# Autodesk Inventor assembly: ASY MSC 800 GILLS
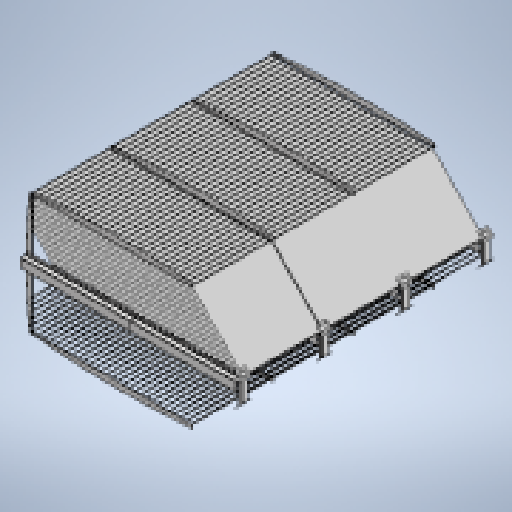
[picture p0: Inventor's stored thumbnail of the model, 512x512]
Saved by Autodesk Inventor 2025.1 (Build 291241020, 241B)
## iProperties
Created: 2024-08-31
Part Number: ASY MSC 800 GILLS
Document SubType Name: Assembly
Designer: pokla
Stock Number: ASY МОО 800 Жабры
Mass: 469810 g
Surface Area: 1.86943e+06 cm^2
Volume: 67870.7 cm^3
Density: 6.92212 g/cm^3
Author: pokla
## Documents named in this file (19)
- C:\Users\user\YandexDisk-badmisterfox\домашниий пк\Inventor\Manturovo\Manturovo_Se-clar\ASY MSC 800 gills.iam
- C:\Users\user\YandexDisk-badmisterfox\домашниий пк\Inventor\Manturovo\Manturovo_Se-clar\MSC 804 sheet gills.ipt
- C:\Users\user\YandexDisk-badmisterfox\домашниий пк\Inventor\Manturovo\Manturovo_Se-clar\MSC 810 pillar gills.ipt
- C:\Users\user\YandexDisk-badmisterfox\домашниий пк\Inventor\Manturovo\Manturovo_Se-clar\MSC 805 sheet gills.ipt
- C:\Users\user\YandexDisk-badmisterfox\домашниий пк\Inventor\Manturovo\Manturovo_Se-clar\MSC 806 sheet gills.ipt
- C:\Users\user\YandexDisk-badmisterfox\домашниий пк\Inventor\Manturovo\Manturovo_Se-clar\MSC 807 sheet gills.ipt
- C:\Users\user\YandexDisk-badmisterfox\домашниий пк\Inventor\Manturovo\Manturovo_Se-clar\MSC 808 sheet gills.ipt
- C:\Users\user\YandexDisk-badmisterfox\домашниий пк\Inventor\Manturovo\Manturovo_Se-clar\MSC 809 sheet gills.ipt
- C:\Users\user\YandexDisk-badmisterfox\домашниий пк\Inventor\Manturovo\Manturovo_Se-clar\MSC 813 wall support gills.ipt
- C:\Users\user\YandexDisk-badmisterfox\домашниий пк\Inventor\Manturovo\Manturovo_Se-clar\MSC 811 pillar gills.ipt
- C:\Users\user\YandexDisk-badmisterfox\домашниий пк\Inventor\Manturovo\Manturovo_Se-clar\MSC 814 string for sheets gills.ipt
- C:\Users\user\YandexDisk-badmisterfox\домашниий пк\Inventor\Manturovo\Manturovo_Se-clar\MSC 812 top support gills.ipt
- C:\Users\user\YandexDisk-badmisterfox\домашниий пк\Inventor\Manturovo\Manturovo_Se-clar\MSC 803 sheet gills.ipt
- C:\Users\user\YandexDisk-badmisterfox\домашниий пк\Inventor\Manturovo\Manturovo_Se-clar\ASY MSC 800.1 gills base.iam
- C:\Users\user\YandexDisk-badmisterfox\домашниий пк\Inventor\Manturovo\Manturovo_Se-clar\MSC 805 sheet gills+.ipt
- C:\Users\user\YandexDisk-badmisterfox\домашниий пк\Inventor\Manturovo\Manturovo_Se-clar\MSC 806 sheet gills+.ipt
- C:\Users\user\YandexDisk-badmisterfox\домашниий пк\Inventor\Manturovo\Manturovo_Se-clar\MSC 807 sheet gills+.ipt
- C:\Users\user\YandexDisk-badmisterfox\домашниий пк\Inventor\Manturovo\Manturovo_Se-clar\MSC 808 sheet gills+.ipt
- C:\Users\user\YandexDisk-badmisterfox\домашниий пк\Inventor\Manturovo\Manturovo_Se-clar\MSC 809 sheet gills+.ipt
## Components (297 placed, 28 different names)
1. MSC 805 sheet gills.ipt:1 — Angle:2, Tangent:8, Tangent:9, Flush:15, Flush:19, Rigid:42
2. MSC 806 sheet gills.ipt:1 — Angle:3, Tangent:10, Tangent:11, Flush:15, Flush:16, Rigid:43
3. MSC 807 sheet gills.ipt:1 — Angle:4, Tangent:12, Tangent:13, Flush:16, Flush:17, Rigid:45
4. MSC 808 sheet gills.ipt:1 — Angle:5, Tangent:17, Tangent:18, Flush:17, Flush:18, Rigid:46
5. MSC 809 sheet gills.ipt:1 — Angle:6, Tangent:19, Tangent:20, Flush:18, Rigid:47
6. MSC 814 string for sheets gills.ipt:1 — Rigid:40
7. MSC 805 sheet gills+.ipt:1 — Rigid:42
8. MSC 806 sheet gills+.ipt:1 — Rigid:43
9. MSC 807 sheet gills+.ipt:1 — Rigid:45
10. MSC 808 sheet gills+.ipt:1 — Rigid:46
11. MSC 809 sheet gills+.ipt:1 — Rigid:47
12. MSC 0203 sheet gills:2 — Rigid:53, Rigid:54
13. MSC 0204 sheet gills:2 — Rigid:54, Rigid:55
14. MSC 0205 sheet gills:2 — Rigid:55, Rigid:56
15. MSC 0206 sheet gills:2 — Rigid:56, Rigid:57
16. MSC 0207 sheet gills:2 — Rigid:57
17. MSC 0103 sheet gills:2
18. MSC 0104 sheet gills:2
19. MSC 0105 sheet gills:2
20. MSC 0106 sheet gills:2
21. MSC 0107 sheet gills:2
22. MSC 814 string for sheets gills.ipt:2 — Rigid:24
23. MSC 814 string for sheets gills.ipt:3
24. MSC 814 string for sheets gills.ipt:4
25. MSC 814 string for sheets gills.ipt:5
26. MSC 814 string for sheets gills.ipt:6
27. MSC 814 string for sheets gills.ipt:7
28. MSC 814 string for sheets gills.ipt:8 — Rigid:12
29. MSC 803 sheet gills.ipt:1 — Rigid:33, Angle:2, Angle:3, Angle:4, Angle:5, Angle:6, Tangent:14, Tangent:15, Tangent:16, Flush:19, Flush:24
30. MSC 804 sheet gills.ipt:1 — Rigid:33
31. MSC 814 string for sheets gills.ipt:9 — Rotational:1
32. MSC 814 string for sheets gills.ipt:10 — Rotational:2, Tangent:23
33. MSC 814 string for sheets gills.ipt:11 — Rotational:3, Tangent:21, Tangent:22
34. MSC 803 sheet gills.ipt:2 — Tangent:21, Tangent:23, Flush:24
35. MSC 804 sheet gills.ipt:2 — Tangent:22
36. MSC 814 string for sheets gills.ipt:12
37. MSC 803 sheet gills.ipt:3
38. MSC 804 sheet gills.ipt:3
39. MSC 814 string for sheets gills.ipt:13
40. MSC 814 string for sheets gills.ipt:14
41. MSC 814 string for sheets gills.ipt:15
42. MSC 803 sheet gills.ipt:4
43. MSC 804 sheet gills.ipt:4
44. MSC 814 string for sheets gills.ipt:16
45. MSC 803 sheet gills.ipt:5
46. MSC 804 sheet gills.ipt:5
47. MSC 814 string for sheets gills.ipt:17
48. MSC 814 string for sheets gills.ipt:18
49. MSC 814 string for sheets gills.ipt:19
50. MSC 803 sheet gills.ipt:6
51. MSC 804 sheet gills.ipt:6
52. MSC 814 string for sheets gills.ipt:20
53. MSC 803 sheet gills.ipt:7
54. MSC 804 sheet gills.ipt:7
55. MSC 814 string for sheets gills.ipt:21
56. MSC 814 string for sheets gills.ipt:22
57. MSC 814 string for sheets gills.ipt:23
58. MSC 803 sheet gills.ipt:8
59. MSC 804 sheet gills.ipt:8
60. MSC 814 string for sheets gills.ipt:24
61. MSC 803 sheet gills.ipt:9
62. MSC 804 sheet gills.ipt:9
63. MSC 814 string for sheets gills.ipt:25
64. MSC 814 string for sheets gills.ipt:26
65. MSC 814 string for sheets gills.ipt:27
66. MSC 803 sheet gills.ipt:10
67. MSC 804 sheet gills.ipt:10
68. MSC 814 string for sheets gills.ipt:28
69. MSC 803 sheet gills.ipt:11
70. MSC 804 sheet gills.ipt:11
71. MSC 814 string for sheets gills.ipt:29
72. MSC 814 string for sheets gills.ipt:30
73. MSC 814 string for sheets gills.ipt:31
74. MSC 803 sheet gills.ipt:12
75. MSC 804 sheet gills.ipt:12
76. MSC 814 string for sheets gills.ipt:32
77. MSC 803 sheet gills.ipt:13
78. MSC 804 sheet gills.ipt:13
79. MSC 814 string for sheets gills.ipt:33
80. MSC 814 string for sheets gills.ipt:34
81. MSC 814 string for sheets gills.ipt:35
82. MSC 803 sheet gills.ipt:14
83. MSC 804 sheet gills.ipt:14
84. MSC 814 string for sheets gills.ipt:36
85. MSC 803 sheet gills.ipt:15
86. MSC 804 sheet gills.ipt:15
87. MSC 814 string for sheets gills.ipt:37
88. MSC 814 string for sheets gills.ipt:38
89. MSC 814 string for sheets gills.ipt:39
90. MSC 803 sheet gills.ipt:16
91. MSC 804 sheet gills.ipt:16
92. MSC 814 string for sheets gills.ipt:40
93. MSC 803 sheet gills.ipt:17
94. MSC 804 sheet gills.ipt:17
95. MSC 814 string for sheets gills.ipt:41
96. MSC 814 string for sheets gills.ipt:42
97. MSC 814 string for sheets gills.ipt:43
98. MSC 803 sheet gills.ipt:18
99. MSC 804 sheet gills.ipt:18
100. MSC 814 string for sheets gills.ipt:44
101. MSC 803 sheet gills.ipt:19
102. MSC 804 sheet gills.ipt:19
103. MSC 814 string for sheets gills.ipt:45
104. MSC 814 string for sheets gills.ipt:46
105. MSC 814 string for sheets gills.ipt:47
106. MSC 803 sheet gills.ipt:20
107. MSC 804 sheet gills.ipt:20
108. MSC 814 string for sheets gills.ipt:48
109. MSC 803 sheet gills.ipt:21
110. MSC 804 sheet gills.ipt:21
111. MSC 814 string for sheets gills.ipt:49
112. MSC 814 string for sheets gills.ipt:50
113. MSC 814 string for sheets gills.ipt:51
114. MSC 803 sheet gills.ipt:22
115. MSC 804 sheet gills.ipt:22
116. MSC 814 string for sheets gills.ipt:52
117. MSC 803 sheet gills.ipt:23
118. MSC 804 sheet gills.ipt:23
119. MSC 814 string for sheets gills.ipt:53
120. MSC 814 string for sheets gills.ipt:54
121. MSC 814 string for sheets gills.ipt:55
122. MSC 803 sheet gills.ipt:24
123. MSC 804 sheet gills.ipt:24
124. MSC 814 string for sheets gills.ipt:56
125. MSC 803 sheet gills.ipt:25
126. MSC 804 sheet gills.ipt:25
127. MSC 814 string for sheets gills.ipt:57
128. MSC 814 string for sheets gills.ipt:58
129. MSC 814 string for sheets gills.ipt:59
130. MSC 803 sheet gills.ipt:26
131. MSC 804 sheet gills.ipt:26
132. MSC 814 string for sheets gills.ipt:60
133. MSC 803 sheet gills.ipt:27
134. MSC 804 sheet gills.ipt:27
135. MSC 814 string for sheets gills.ipt:61
136. MSC 814 string for sheets gills.ipt:62
137. MSC 814 string for sheets gills.ipt:63
138. MSC 803 sheet gills.ipt:28
139. MSC 804 sheet gills.ipt:28
140. MSC 814 string for sheets gills.ipt:64
141. MSC 803 sheet gills.ipt:29
142. MSC 804 sheet gills.ipt:29
143. MSC 814 string for sheets gills.ipt:65
144. MSC 814 string for sheets gills.ipt:66
145. MSC 814 string for sheets gills.ipt:67
146. MSC 803 sheet gills.ipt:30
147. MSC 804 sheet gills.ipt:30
148. MSC 814 string for sheets gills.ipt:68
149. MSC 803 sheet gills.ipt:31
150. MSC 804 sheet gills.ipt:31
151. MSC 814 string for sheets gills.ipt:69
152. MSC 814 string for sheets gills.ipt:70
153. MSC 814 string for sheets gills.ipt:71
154. MSC 803 sheet gills.ipt:32
155. MSC 804 sheet gills.ipt:32
156. MSC 814 string for sheets gills.ipt:72
157. MSC 803 sheet gills.ipt:33
158. MSC 804 sheet gills.ipt:33
159. MSC 814 string for sheets gills.ipt:73
160. MSC 814 string for sheets gills.ipt:74
161. MSC 814 string for sheets gills.ipt:75
162. MSC 803 sheet gills.ipt:34
163. MSC 804 sheet gills.ipt:34
164. MSC 814 string for sheets gills.ipt:76
165. MSC 803 sheet gills.ipt:35
166. MSC 804 sheet gills.ipt:35
167. MSC 814 string for sheets gills.ipt:77
168. MSC 814 string for sheets gills.ipt:78
169. MSC 814 string for sheets gills.ipt:79
170. MSC 803 sheet gills.ipt:36
171. MSC 804 sheet gills.ipt:36
172. MSC 814 string for sheets gills.ipt:80
173. MSC 803 sheet gills.ipt:37
174. MSC 804 sheet gills.ipt:37
175. MSC 814 string for sheets gills.ipt:81
176. MSC 814 string for sheets gills.ipt:82
177. MSC 814 string for sheets gills.ipt:83
178. MSC 803 sheet gills.ipt:38
179. MSC 804 sheet gills.ipt:38
180. MSC 814 string for sheets gills.ipt:84
181. MSC 803 sheet gills.ipt:39
182. MSC 804 sheet gills.ipt:39
183. MSC 814 string for sheets gills.ipt:85
184. MSC 814 string for sheets gills.ipt:86
185. MSC 814 string for sheets gills.ipt:87
186. MSC 803 sheet gills.ipt:40
187. MSC 804 sheet gills.ipt:40
188. MSC 814 string for sheets gills.ipt:88
189. MSC 803 sheet gills.ipt:41
190. MSC 804 sheet gills.ipt:41
191. MSC 814 string for sheets gills.ipt:89
192. MSC 814 string for sheets gills.ipt:90
193. MSC 814 string for sheets gills.ipt:91
194. MSC 803 sheet gills.ipt:42
195. MSC 804 sheet gills.ipt:42
196. MSC 814 string for sheets gills.ipt:92
197. MSC 803 sheet gills.ipt:43
198. MSC 804 sheet gills.ipt:43
199. MSC 814 string for sheets gills.ipt:93
200. MSC 814 string for sheets gills.ipt:94
201. MSC 814 string for sheets gills.ipt:95
202. MSC 803 sheet gills.ipt:44
203. MSC 804 sheet gills.ipt:44
204. MSC 814 string for sheets gills.ipt:96
205. MSC 803 sheet gills.ipt:45
206. MSC 804 sheet gills.ipt:45
207. MSC 814 string for sheets gills.ipt:97
208. MSC 814 string for sheets gills.ipt:98
209. MSC 814 string for sheets gills.ipt:99
210. MSC 803 sheet gills.ipt:46
211. MSC 804 sheet gills.ipt:46
212. MSC 814 string for sheets gills.ipt:100
213. MSC 803 sheet gills.ipt:47
214. MSC 804 sheet gills.ipt:47
215. MSC 814 string for sheets gills.ipt:101
216. MSC 814 string for sheets gills.ipt:102
217. MSC 814 string for sheets gills.ipt:103
218. MSC 803 sheet gills.ipt:48
219. MSC 804 sheet gills.ipt:48
220. MSC 814 string for sheets gills.ipt:104
221. MSC 803 sheet gills.ipt:49
222. MSC 804 sheet gills.ipt:49
223. MSC 814 string for sheets gills.ipt:105
224. MSC 814 string for sheets gills.ipt:106
225. MSC 814 string for sheets gills.ipt:107
226. MSC 803 sheet gills.ipt:50
227. MSC 804 sheet gills.ipt:50
228. MSC 814 string for sheets gills.ipt:108
229. MSC 803 sheet gills.ipt:51
230. MSC 804 sheet gills.ipt:51
231. MSC 814 string for sheets gills.ipt:109
232. MSC 814 string for sheets gills.ipt:110
233. MSC 814 string for sheets gills.ipt:111
234. MSC 803 sheet gills.ipt:52
235. MSC 804 sheet gills.ipt:52
236. MSC 814 string for sheets gills.ipt:112
237. MSC 803 sheet gills.ipt:53
238. MSC 804 sheet gills.ipt:53
239. MSC 814 string for sheets gills.ipt:113
240. MSC 814 string for sheets gills.ipt:114
241. MSC 814 string for sheets gills.ipt:115
242. MSC 803 sheet gills.ipt:54
243. MSC 804 sheet gills.ipt:54
244. MSC 814 string for sheets gills.ipt:116
245. MSC 803 sheet gills.ipt:55
246. MSC 804 sheet gills.ipt:55
247. MSC 814 string for sheets gills.ipt:117
248. MSC 814 string for sheets gills.ipt:118
249. MSC 814 string for sheets gills.ipt:119
250. MSC 803 sheet gills.ipt:56
251. MSC 804 sheet gills.ipt:56
252. MSC 814 string for sheets gills.ipt:120
253. MSC 803 sheet gills.ipt:57
254. MSC 804 sheet gills.ipt:57
255. MSC 814 string for sheets gills.ipt:121
256. MSC 814 string for sheets gills.ipt:122
257. MSC 814 string for sheets gills.ipt:123
258. MSC 803 sheet gills.ipt:58 — Rigid:53
259. MSC 804 sheet gills.ipt:58
260. MSC 813 wall support gills.ipt:1 — Rigid:12, Rigid:30, Tangent:14, Tangent:15
261. MSC 812 top support gills.ipt:1 — Rigid:28, Rigid:30, Tangent:8, Tangent:9, Tangent:10, Tangent:11, Tangent:12, Tangent:13, Tangent:17, Tangent:18, Tangent:19, Tangent:20, Rigid:40, Rigid:44
262. MSC 811 pillar gills.ipt:1 — Rigid:28, Rigid:29
263. MSC 812 top support gills.ipt:2 — Rigid:24, Rigid:29, Rigid:31
264. MSC 813 wall support gills.ipt:2 — Rigid:31, Rotational:3
265. MSC 810 pillar gills.ipt:1 — Rotational:1, Rotational:2, Tangent:16
266. ASY MSC 800.1 gills base.iam:1 [sub-assembly]
267. MSC 813 wall support gills.ipt:3
268. MSC 812 top support gills.ipt:3
269. MSC 811 pillar gills.ipt:2
270. MSC 812 top support gills.ipt:4
271. MSC 813 wall support gills.ipt:4
272. MSC 810 pillar gills.ipt:2
273. ASY MSC 800.1 gills base.iam:2 [sub-assembly]
274. MSC 813 wall support gills.ipt:5
275. MSC 812 top support gills.ipt:5
276. MSC 811 pillar gills.ipt:3
277. MSC 812 top support gills.ipt:6
278. MSC 813 wall support gills.ipt:6
279. MSC 810 pillar gills.ipt:3
280. ASY MSC 800.1 gills base.iam:3 [sub-assembly]
281. MSC 813 wall support gills.ipt:7
282. MSC 812 top support gills.ipt:7
283. MSC 811 pillar gills.ipt:4 — Rotational:4
284. MSC 812 top support gills.ipt:8
285. MSC 813 wall support gills.ipt:8
286. MSC 810 pillar gills.ipt:4
287. ASY MSC 800.1 gills base.iam:4 [sub-assembly]
288. MSC 814 string for sheets gills.ipt:124 — Rotational:4
289. MSC 814 string for sheets gills.ipt:125
290. MSC 814 string for sheets gills.ipt:126
291. MSC 814 string for sheets gills.ipt:127
292. MSC 814 string for sheets gills.ipt:128
293. MSC 814 string for sheets gills.ipt:129 — Rigid:44
294. MSC 814 string for sheets gills.ipt:130
295. MSC 814 string for sheets gills.ipt:131
296. MSC 814 string for sheets gills.ipt:132
297. MSC 814 string for sheets gills.ipt:133
## Component patterns: (6 elements, first: MSC 814 string for sheets gills.ipt:2), (29 elements, first: MSC 814 string for sheets gills.ipt:8 + MSC 803 sheet gills.ipt:1 + MSC 804 sheet gills.ipt:1 + MSC 814 string for sheets gills.ipt:9 + MSC 814 string for sheets gills.ipt:10 + MSC 814 string for sheets gills.ipt:11 + MSC 803 sheet gills.ipt:2 + MSC 804 sheet gills.ipt:2), (4 elements, first: MSC 813 wall support gills.ipt:1 + MSC 812 top support gills.ipt:1 + MSC 811 pillar gills.ipt:1 + MSC 812 top support gills.ipt:2 + MSC 813 wall support gills.ipt:2 + MSC 810 pillar gills.ipt:1 + ASY MSC 800.1 gills base.iam:1), (5 elements, first: MSC 814 string for sheets gills.ipt:124), (5 elements, first: MSC 814 string for sheets gills.ipt:129)
## Relationships (64: WeldJoint 26, Tangent 16, Flush 10, Angle 5, RevoluteJoint 4, Mate 3)
- [WeldJoint]: MSC 811 pillar gills.ipt:1 ↔ MSC 810 pillar gills.ipt:1
- [Flush]: MSC 810 pillar gills.ipt:1 ↔ ASY MSC 800.1 gills base.iam:1
- [Mate]: MSC 810 pillar gills.ipt:1 ↔ ASY MSC 800.1 gills base.iam:1
- [Flush] (5 mm): MSC 810 pillar gills.ipt:1 ↔ ASY MSC 800.1 gills base.iam:1
- Rigid:12 [WeldJoint] (-5 mm): MSC 814 string for sheets gills.ipt:8 ↔ MSC 813 wall support gills.ipt:1
- [Mate]: ASY MSC 800.1 gills base.iam:1
- [Mate]: ASY MSC 800.1 gills base.iam:1
- [Flush]: ASY MSC 800.1 gills base.iam:1
- Rigid:24 [WeldJoint] (-5 mm): MSC 814 string for sheets gills.ipt:2 ↔ MSC 812 top support gills.ipt:2
- Rigid:28 [WeldJoint]: MSC 812 top support gills.ipt:1 ↔ MSC 811 pillar gills.ipt:1
- Rigid:29 [WeldJoint]: MSC 811 pillar gills.ipt:1 ↔ MSC 812 top support gills.ipt:2
- Rigid:30 [WeldJoint]: MSC 813 wall support gills.ipt:1 ↔ MSC 812 top support gills.ipt:1
- Rigid:31 [WeldJoint]: MSC 812 top support gills.ipt:2 ↔ MSC 813 wall support gills.ipt:2
- Rotational:1 [RevoluteJoint] (5 mm): MSC 814 string for sheets gills.ipt:9 ↔ MSC 810 pillar gills.ipt:1
- Rotational:2 [RevoluteJoint] (-5 mm): MSC 814 string for sheets gills.ipt:10 ↔ MSC 810 pillar gills.ipt:1
- Rigid:33 [WeldJoint] (-10 mm): MSC 803 sheet gills.ipt:1 ↔ MSC 804 sheet gills.ipt:1
- Angle:2 (0 deg): MSC 805 sheet gills.ipt:1 ↔ MSC 803 sheet gills.ipt:1
- Angle:3 (0 deg): MSC 806 sheet gills.ipt:1 ↔ MSC 803 sheet gills.ipt:1
- Angle:4 (0 deg): MSC 807 sheet gills.ipt:1 ↔ MSC 803 sheet gills.ipt:1
- Angle:5 (0 deg): MSC 808 sheet gills.ipt:1 ↔ MSC 803 sheet gills.ipt:1
- Angle:6 (0 deg): MSC 809 sheet gills.ipt:1 ↔ MSC 803 sheet gills.ipt:1
- Tangent:8: MSC 805 sheet gills.ipt:1 ↔ MSC 812 top support gills.ipt:1
- Tangent:9: MSC 805 sheet gills.ipt:1 ↔ MSC 812 top support gills.ipt:1
- Tangent:10: MSC 806 sheet gills.ipt:1 ↔ MSC 812 top support gills.ipt:1
- Tangent:11: MSC 806 sheet gills.ipt:1 ↔ MSC 812 top support gills.ipt:1
- Tangent:12: MSC 807 sheet gills.ipt:1 ↔ MSC 812 top support gills.ipt:1
- Tangent:13: MSC 807 sheet gills.ipt:1 ↔ MSC 812 top support gills.ipt:1
- Tangent:14: MSC 803 sheet gills.ipt:1 ↔ MSC 813 wall support gills.ipt:1
- Tangent:15: MSC 803 sheet gills.ipt:1 ↔ MSC 813 wall support gills.ipt:1
- Tangent:16: MSC 803 sheet gills.ipt:1 ↔ MSC 810 pillar gills.ipt:1
- Tangent:17: MSC 808 sheet gills.ipt:1 ↔ MSC 812 top support gills.ipt:1
- Tangent:18: MSC 808 sheet gills.ipt:1 ↔ MSC 812 top support gills.ipt:1
- Tangent:19: MSC 809 sheet gills.ipt:1 ↔ MSC 812 top support gills.ipt:1
- Tangent:20: MSC 809 sheet gills.ipt:1 ↔ MSC 812 top support gills.ipt:1
- Flush:15: MSC 805 sheet gills.ipt:1 ↔ MSC 806 sheet gills.ipt:1
- Flush:16: MSC 806 sheet gills.ipt:1 ↔ MSC 807 sheet gills.ipt:1
- Flush:17: MSC 807 sheet gills.ipt:1 ↔ MSC 808 sheet gills.ipt:1
- Flush:18: MSC 808 sheet gills.ipt:1 ↔ MSC 809 sheet gills.ipt:1
- Flush:19: MSC 805 sheet gills.ipt:1 ↔ MSC 803 sheet gills.ipt:1
- Rigid:40 [WeldJoint] (5 mm): MSC 814 string for sheets gills.ipt:1 ↔ MSC 812 top support gills.ipt:1
- Rotational:3 [RevoluteJoint] (-5 mm): MSC 814 string for sheets gills.ipt:11 ↔ MSC 813 wall support gills.ipt:2
- [WeldJoint] (-10 mm): MSC 803 sheet gills.ipt:2 ↔ MSC 804 sheet gills.ipt:2
- Tangent:21: MSC 814 string for sheets gills.ipt:11 ↔ MSC 803 sheet gills.ipt:2
- Tangent:22: MSC 814 string for sheets gills.ipt:11 ↔ MSC 804 sheet gills.ipt:2
- Tangent:23: MSC 814 string for sheets gills.ipt:10 ↔ MSC 803 sheet gills.ipt:2
- Flush:24: MSC 803 sheet gills.ipt:1 ↔ MSC 803 sheet gills.ipt:2
- Rigid:42 [WeldJoint] (-10 mm): MSC 805 sheet gills.ipt:1 ↔ MSC 805 sheet gills+.ipt:1
- Rotational:4 [RevoluteJoint] (22 mm): MSC 811 pillar gills.ipt:4 ↔ MSC 814 string for sheets gills.ipt:124
- Rigid:43 [WeldJoint] (-10 mm): MSC 806 sheet gills.ipt:1 ↔ MSC 806 sheet gills+.ipt:1
- Rigid:44 [WeldJoint] (5 mm): MSC 812 top support gills.ipt:1 ↔ MSC 814 string for sheets gills.ipt:129
- Rigid:45 [WeldJoint] (-10 mm): MSC 807 sheet gills.ipt:1 ↔ MSC 807 sheet gills+.ipt:1
- Rigid:46 [WeldJoint] (-10 mm): MSC 808 sheet gills.ipt:1 ↔ MSC 808 sheet gills+.ipt:1
- Rigid:47 [WeldJoint] (-10 mm): MSC 809 sheet gills.ipt:1 ↔ MSC 809 sheet gills+.ipt:1
- [Flush]: MSC 0203 sheet gills:2 ↔ MSC 0204 sheet gills:2
- [WeldJoint] (-10 mm): MSC 0203 sheet gills:2 ↔ MSC 0103 sheet gills:2
- [WeldJoint] (-10 mm): MSC 0204 sheet gills:2 ↔ MSC 0104 sheet gills:2
- [WeldJoint] (-10 mm): MSC 0205 sheet gills:2 ↔ MSC 0105 sheet gills:2
- [WeldJoint] (-10 mm): MSC 0206 sheet gills:2 ↔ MSC 0106 sheet gills:2
- [WeldJoint] (-10 mm): MSC 0207 sheet gills:2 ↔ MSC 0107 sheet gills:2
- Rigid:53 [WeldJoint] (50 mm): MSC 0203 sheet gills:2 ↔ MSC 803 sheet gills.ipt:58
- Rigid:54 [WeldJoint] (50 mm): MSC 0203 sheet gills:2 ↔ MSC 0204 sheet gills:2
- Rigid:55 [WeldJoint] (50 mm): MSC 0204 sheet gills:2 ↔ MSC 0205 sheet gills:2
- Rigid:56 [WeldJoint] (50 mm): MSC 0205 sheet gills:2 ↔ MSC 0206 sheet gills:2
- Rigid:57 [WeldJoint] (50 mm): MSC 0206 sheet gills:2 ↔ MSC 0207 sheet gills:2
## Named parameters: d269_d176 = -10 mm, d291_d281 = -10 mm, d292_d287 = -10 mm, d293_d289 = -10 mm, d294_d290 = -10 mm, d295_d274 = -10 mm, d296_d202 = 0 mm
